# Autodesk Inventor assembly: Tension_Thingy_v2
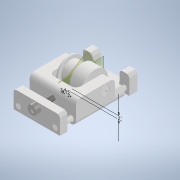
[picture p0: Inventor's stored thumbnail of the model, 180x180]
Saved by Autodesk Inventor 2022 (Build 260153000, 153)
## iProperties
Created: 2023-07-28
Part Number: Tension_Thingy_v2
Document SubType Name: Assembly
Designer: aewalder
Author: aewalder
## Documents named in this file (8)
- C:\Users\AEWALDER\Documents\Inventor\03_CurrentProjects\MasterThesis\PSM_V1_Rillenkugellager\Tension_Thingy_v2.iam
- C:\Users\AEWALDER\Documents\Inventor\03_CurrentProjects\MasterThesis\PSM_V1_Rillenkugellager\Tension_Bock.ipt
- C:\Users\AEWALDER\Documents\Inventor\03_CurrentProjects\MasterThesis\PSM_V1_Rillenkugellager\Spannvorrichtung_Riemen.ipt
- C:\Users\AEWALDER\Documents\Inventor\03_CurrentProjects\MasterThesis\PSM_V1_Rillenkugellager\ContentCenter\en-US\DIN EN ISO 4032\DIN EN ISO 4032 - M3.ipt
- C:\Users\AEWALDER\Documents\Inventor\03_CurrentProjects\MasterThesis\PSM_V1_Rillenkugellager\Riemenscheibe.ipt
- C:\Users\AEWALDER\Documents\Inventor\03_CurrentProjects\MasterThesis\PSM_V1_Rillenkugellager\Fuehrungsschienen_Tension.ipt
- C:\Users\AEWALDER\Documents\Inventor\03_CurrentProjects\MasterThesis\PSM_V1_Rillenkugellager\ContentCenter\en-US\ISO 4762(1)\DIN EN ISO 4762 - M3 x 16.ipt
- C:\Users\AEWALDER\Documents\Inventor\03_CurrentProjects\MasterThesis\PSM_V1_Rillenkugellager\Riemenscheibe_Welle_Tension.ipt
## Components (8 placed, 7 different names)
1. Tension_Bock:1 — Mate:1, Mate:2, Mate:3, Flush:1, Flush:2, Flush:3, Flush:5, Mate:8, Flush:6, Mate:10
2. Spannvorrichtung_Riemen:1 — Mate:1, Mate:2, Mate:4, Mate:5, Flush:4, Mate:7, Mate:11, Flush:7
3. DIN EN ISO 4032 M3:1 — Mate:3, Mate:4, Mate:9
4. Riemenscheibe:1 — Mate:6, Flush:4
5. Fuehrungsschienen_Tension:1 — Mate:7, Flush:5
6. Fuehrungsschienen_Tension:2 — Mate:8, Flush:6
7. DIN EN ISO 4762 M3 x 16:1 — Mate:9, Mate:10
8. Riemenscheibe_Welle_Tension:1 — Mate:11, Flush:7
## Relationships (18: Mate 11, Flush 7)
- Mate:1: Tension_Bock:1 ↔ Spannvorrichtung_Riemen:1
- Mate:2: Tension_Bock:1 ↔ Spannvorrichtung_Riemen:1
- Mate:3: Tension_Bock:1 ↔ DIN EN ISO 4032 M3:1
- Flush:1: Tension_Bock:1
- Flush:2: Tension_Bock:1
- Flush:3: Tension_Bock:1
- Mate:4: Spannvorrichtung_Riemen:1 ↔ DIN EN ISO 4032 M3:1
- Mate:5: Spannvorrichtung_Riemen:1
- Mate:6: Riemenscheibe:1
- Flush:4: Spannvorrichtung_Riemen:1 ↔ Riemenscheibe:1
- Mate:7: Spannvorrichtung_Riemen:1 ↔ Fuehrungsschienen_Tension:1
- Flush:5: Tension_Bock:1 ↔ Fuehrungsschienen_Tension:1
- Mate:8: Tension_Bock:1 ↔ Fuehrungsschienen_Tension:2
- Flush:6: Tension_Bock:1 ↔ Fuehrungsschienen_Tension:2
- Mate:9: DIN EN ISO 4032 M3:1 ↔ DIN EN ISO 4762 M3 x 16:1
- Mate:10: Tension_Bock:1 ↔ DIN EN ISO 4762 M3 x 16:1
- Mate:11: Spannvorrichtung_Riemen:1 ↔ Riemenscheibe_Welle_Tension:1
- Flush:7: Spannvorrichtung_Riemen:1 ↔ Riemenscheibe_Welle_Tension:1
